# Autodesk Inventor assembly: bike
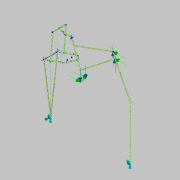
[picture p0: Inventor's stored thumbnail of the model, 180x180]
Saved by Autodesk Inventor 2021 (Build 250183000, 183)
## iProperties
RuleStatus: InUse
Created: 2020-04-29
Part Number: bike
Document SubType Name: Assembly
Designer: Hannah
Mass: 8583.94 g
Surface Area: 13590.5 cm^2
Volume: 2798.24 cm^3
Density: 3.06762 g/cm^3
Author: Hannah
## Documents named in this file (29)
- \\Mac\Home\Documents\GitHub\AdjustaBike-2.0\CAD\bike.iam
- \\Mac\Home\Documents\GitHub\AdjustaBike-2.0\CAD\prelim bike geo.ipt
- \\Mac\Home\Documents\GitHub\AdjustaBike-2.0\CAD\bottom bracket.ipt
- \\Mac\Home\Documents\GitHub\AdjustaBike-2.0\CAD\L10-7.ipt
- \\Mac\Home\Documents\GitHub\AdjustaBike-2.0\CAD\tube-07.ipt
- \\Mac\Home\Documents\GitHub\AdjustaBike-2.0\CAD\tube-08.ipt
- \\Mac\Home\Documents\GitHub\AdjustaBike-2.0\CAD\tube-09.ipt
- \\Mac\Home\Documents\GitHub\AdjustaBike-2.0\CAD\tube-11.ipt
- \\Mac\Home\Documents\GitHub\AdjustaBike-2.0\CAD\tube-12.ipt
- \\Mac\Home\Documents\GitHub\AdjustaBike-2.0\CAD\329-7.ipt
- \\Mac\Home\Documents\GitHub\AdjustaBike-2.0\CAD\head tube.ipt
- \\Mac\Home\Documents\GitHub\AdjustaBike-2.0\CAD\LM50-7.ipt
- \\Mac\Home\Documents\GitHub\AdjustaBike-2.0\CAD\LF50-6.ipt
- \\Mac\Home\Documents\GitHub\AdjustaBike-2.0\CAD\55-7.ipt
- \\Mac\Home\Documents\GitHub\AdjustaBike-2.0\CAD\L21-7.ipt
- \\Mac\Home\Documents\GitHub\AdjustaBike-2.0\CAD\tube-13.ipt
- \\Mac\Home\Documents\GitHub\AdjustaBike-2.0\CAD\LF50-7.ipt
- \\Mac\Home\Documents\GitHub\AdjustaBike-2.0\CAD\L10-6.ipt
- \\Mac\Home\Documents\GitHub\AdjustaBike-2.0\CAD\tube-14.ipt
- \\Mac\Home\Documents\GitHub\AdjustaBike-2.0\CAD\L114-6.ipt
- \\Mac\Home\Documents\GitHub\AdjustaBike-2.0\CAD\saddle.ipt
- \\Mac\Home\Documents\GitHub\AdjustaBike-2.0\CAD\M51-5.ipt
- \\Mac\Home\Documents\GitHub\AdjustaBike-2.0\CAD\link.ipt
- \\Mac\Home\Documents\GitHub\AdjustaBike-2.0\CAD\LM51-7.ipt
- \\Mac\Home\Documents\GitHub\AdjustaBike-2.0\CAD\main frame.ipt
- \\Mac\Home\Documents\GitHub\AdjustaBike-2.0\CAD\projectile.ipt
- \\Mac\Home\Documents\GitHub\AdjustaBike-2.0\CAD\dummy fork.ipt
- \\Mac\Home\Documents\GitHub\AdjustaBike-2.0\CAD\seatstays.ipt
- \\Mac\Home\Documents\GitHub\AdjustaBike-2.0\CAD\wheels.ipt
## Components (43 placed, 28 different names)
1. prelim bike geo:1 — Mate:1, Mate:2, Angle:1, Mate:41, Mate:140, Mate:149
2. main frame:1 — Mate:115, Mate:116, Mate:117, Mate:118, Mate:119, Mate:120, Mate:121, Mate:122, Mate:123, Mate:124, Mate:125, Mate:126, Mate:127, Mate:128, Mate:129, Mate:131, Mate:132, Mate:133, Mate:134, Mate:135, Mate:136, Mate:137, Mate:138, Mate:139, Mate:140, Mate:141, Mate:142, Mate:144, Flush:117, Flush:118, Flush:119, Flush:120, Flush:121, Flush:122, Flush:123, Flush:124, Flush:125
3. seatstays:1 — Flush:120, Flush:121, Flush:122, Mate:147, Mate:148
4. dummy fork:1 — Flush:117, Flush:118, Flush:119, Mate:149
5. projectile:1 — Mate:142, Mate:143, Mate:144, Mate:146
6. wheels:1 — Flush:123, Flush:124, Flush:125
7. bottom bracket:1 — Mate:4, Flush:1, Mate:5, Mate:6, Tangent:1, Mate:128, Mate:132, Mate:133
8. L10-7:1 — Mate:6, Flush:2, Mate:7, Mate:9
9. seat tube — Mate:7, Tangent:1, Flush:9, Angle:2, Mate:8, Angle:5, Mate:17, Tangent:7, Tangent:8, Mate:28, Mate:52, Flush:21, Mate:106, Mate:117
10. down tube — Flush:10, Angle:3, Tangent:2, Mate:11, Tangent:3, Angle:4, Mate:12, Mate:116
11. top tube — Mate:16, Tangent:4, Mate:18, Mate:115
12. seatstay:2 — Mate:45, Mate:47, Mate:82, Tangent:9, Mate:124
13. spacer:1 — Tangent:8, Mate:55, Mate:57, Mate:61, Mate:120
14. spacer:2 — Tangent:7, Mate:54, Mate:56, Mate:63, Mate:119
15. 329-7:1 — Mate:8, Mate:9, Mate:10, Angle:3, Tangent:2, Mate:11, Mate:53
16. 329-7:2 — Tangent:3, Angle:4, Mate:12, Mate:13, Mate:14, Flush:11
17. head tube:1 — Mate:14, Flush:11, Flush:12, Angle:5, Mate:15, Flush:13, Tangent:4, Mate:118, Mate:131
18. L10-7:2 — Mate:17, Mate:18
19. L10-7:3 — Mate:15, Flush:13, Flush:14, Mate:16, Mate:129
20. LM51-7:1 — Mate:28, Flush:16, Mate:69, Flush:20, Flush:21, Flush:22, Mate:107, Mate:110, Mate:111, Mate:112, Mate:113, Mate:114, Mate:138, Mate:139
21. LF50-6:2 — Mate:45, Mate:47, Angle:11, Mate:83, Flush:85
22. 55-7:1 — Mate:56, Mate:59, Mate:63, Mate:64
23. 55-7:2 — Mate:57, Mate:58, Mate:61, Mate:62
24. L21-7:1 — Mate:52, Mate:53, Mate:54, Mate:55, Mate:60
25. tube-13:1 — Mate:58, Mate:62, Angle:12, Mate:75, Mate:77, Mate:122
26. tube-13:2 — Mate:59, Mate:64, Angle:13, Mate:74, Mate:76, Mate:121
27. LF50-6:3 — Mate:69, Flush:20, Mate:98, Mate:99, Mate:108, Mate:109, Mate:126, Mate:141
28. LF50-7:1 — Mate:76, Mate:79, Mate:85, Mate:94, Mate:127, Mate:134
29. LF50-7:2 — Mate:77, Mate:78, Mate:85, Mate:86, Mate:135
30. LM50-7:3 — Mate:75, Mate:83, Flush:85, Mate:86
31. LM50-7:4 — Mate:74, Mate:94, Mate:95, Mate:96
32. L10-6:1 — Mate:82, Mate:89, Mate:137
33. tube-14:1 — Mate:89, Mate:90, Mate:92, Mate:100, Tangent:9, Mate:125, Mate:136, Mate:147, Mate:148
34. seatstay:1 — Mate:91, Mate:93, Mate:97, Mate:123
35. L10-6:3 — Mate:91, Mate:92
36. LF50-6:4 — Mate:93, Mate:95, Mate:96, Mate:97
37. L114-6:1 — Mate:98, Mate:99, Mate:100
38. saddle:1 — Mate:106, Flush:116
39. M51-5:1
40. link:1 — Mate:107, Mate:109
41. link:2 — Mate:111, Mate:113
42. link:3 — Mate:108, Mate:112
43. link:4 — Mate:110, Mate:114
## Relationships (143: Mate 105, Flush 23, Angle 8, Tangent 7)
- Mate:1: prelim bike geo:1
- Mate:2: prelim bike geo:1
- Mate:3
- Mate:4: bottom bracket:1
- Flush:1: bottom bracket:1
- Angle:1 (0 deg): prelim bike geo:1
- Mate:5: bottom bracket:1
- Mate:6: bottom bracket:1 ↔ L10-7:1
- Flush:2: L10-7:1
- Mate:7: L10-7:1 ↔ seat tube
- Tangent:1: bottom bracket:1 ↔ seat tube
- Flush:9: seat tube
- Angle:2 (-70 deg): seat tube
- Flush:10: down tube
- Mate:8: seat tube ↔ 329-7:1
- Mate:9 (5 mm): L10-7:1 ↔ 329-7:1
- Mate:10: 329-7:1
- Angle:3 (72 deg): down tube ↔ 329-7:1
- Tangent:2: down tube ↔ 329-7:1
- Mate:11: down tube ↔ 329-7:1
- Tangent:3: down tube ↔ 329-7:2
- Angle:4 (0 deg): down tube ↔ 329-7:2
- Mate:12: down tube ↔ 329-7:2
- Mate:13: 329-7:2
- Mate:14: 329-7:2 ↔ head tube:1
- Flush:11: 329-7:2 ↔ head tube:1
- Flush:12: head tube:1
- Angle:5 (0 deg): seat tube ↔ head tube:1
- Mate:15: head tube:1 ↔ L10-7:3
- Flush:13: head tube:1 ↔ L10-7:3
- Flush:14: L10-7:3
- Mate:16: top tube ↔ L10-7:3
- Tangent:4: top tube ↔ head tube:1
- Mate:17: seat tube ↔ L10-7:2
- Mate:18: top tube ↔ L10-7:2
- Tangent:7: seat tube ↔ spacer:2
- Tangent:8: seat tube ↔ spacer:1
- Mate:28: seat tube ↔ LM51-7:1
- Flush:16: LM51-7:1
- Mate:41: prelim bike geo:1
- Mate:45: seatstay:2 ↔ LF50-6:2
- Mate:47: seatstay:2 ↔ LF50-6:2
- Angle:11 (0 deg): LF50-6:2
- Mate:52: seat tube ↔ L21-7:1
- Mate:53 (5 mm): 329-7:1 ↔ L21-7:1
- Mate:54: spacer:2 ↔ L21-7:1
- Mate:55: spacer:1 ↔ L21-7:1
- Mate:56: spacer:2 ↔ 55-7:1
- Mate:57: spacer:1 ↔ 55-7:2
- Mate:58: 55-7:2 ↔ tube-13:1
- Mate:59: 55-7:1 ↔ tube-13:2
- Mate:60: L21-7:1
- Mate:61 (-30 mm): spacer:1 ↔ 55-7:2
- Mate:62 (-30 mm): 55-7:2 ↔ tube-13:1
- Mate:63 (-30 mm): spacer:2 ↔ 55-7:1
- Mate:64 (-30 mm): 55-7:1 ↔ tube-13:2
- Angle:12 (0 deg): tube-13:1
- Angle:13 (0 deg): tube-13:2
- Mate:69: LM51-7:1 ↔ LF50-6:3
- Flush:20: LM51-7:1 ↔ LF50-6:3
- Flush:21: seat tube ↔ LM51-7:1
- Mate:74: tube-13:2 ↔ LM50-7:4
- Mate:75: tube-13:1 ↔ LM50-7:3
- Mate:76: tube-13:2 ↔ LF50-7:1
- Mate:77: tube-13:1 ↔ LF50-7:2
- Mate:78: LF50-7:2
- Mate:79: LF50-7:1
- Flush:22: LM51-7:1
- Mate:82: seatstay:2 ↔ L10-6:1
- Mate:83: LF50-6:2 ↔ LM50-7:3
- Flush:85: LF50-6:2 ↔ LM50-7:3
- Mate:85: LF50-7:1 ↔ LF50-7:2
- Mate:86 (5 mm): LF50-7:2 ↔ LM50-7:3
- Mate:89: L10-6:1 ↔ tube-14:1
- Mate:90: tube-14:1
- Mate:91: seatstay:1 ↔ L10-6:3
- Mate:92: tube-14:1 ↔ L10-6:3
- Mate:93: seatstay:1 ↔ LF50-6:4
- Mate:94 (5 mm): LF50-7:1 ↔ LM50-7:4
- Mate:95: LM50-7:4 ↔ LF50-6:4
- Mate:96: LM50-7:4 ↔ LF50-6:4
- Mate:97: seatstay:1 ↔ LF50-6:4
- Mate:98: LF50-6:3 ↔ L114-6:1
- Mate:99: LF50-6:3 ↔ L114-6:1
- Mate:100: tube-14:1 ↔ L114-6:1
- Tangent:9: seatstay:2 ↔ tube-14:1
- [Mate]: saddle:1 ↔ M51-5:1
- [Mate]: M51-5:1 ↔ link:3
- [Mate]: M51-5:1 ↔ link:4
- [Mate]: M51-5:1 ↔ link:2
- [Mate]: M51-5:1 ↔ link:1
- Mate:106: seat tube ↔ saddle:1
- Mate:107: LM51-7:1 ↔ link:1
- Mate:108: LF50-6:3 ↔ link:3
- Mate:109: LF50-6:3 ↔ link:1
- Mate:110: LM51-7:1 ↔ link:4
- Mate:111: LM51-7:1 ↔ link:2
- Mate:112: LM51-7:1 ↔ link:3
- Mate:113: LM51-7:1 ↔ link:2
- Mate:114: LM51-7:1 ↔ link:4
- Flush:116: saddle:1
- Mate:115: main frame:1 ↔ top tube
- Mate:116: main frame:1 ↔ down tube
- Mate:117: main frame:1 ↔ seat tube
- Mate:118: main frame:1 ↔ head tube:1
- Mate:119: main frame:1 ↔ spacer:2
- Mate:120: main frame:1 ↔ spacer:1
- Mate:121: main frame:1 ↔ tube-13:2
- Mate:122: main frame:1 ↔ tube-13:1
- Mate:123: main frame:1 ↔ seatstay:1
- Mate:124: main frame:1 ↔ seatstay:2
- Mate:125: main frame:1 ↔ tube-14:1
- Mate:126: main frame:1 ↔ LF50-6:3
- Mate:127: main frame:1 ↔ LF50-7:1
- Mate:128: main frame:1 ↔ bottom bracket:1
- Mate:129: main frame:1 ↔ L10-7:3
- Mate:131: main frame:1 ↔ head tube:1
- Mate:132: main frame:1 ↔ bottom bracket:1
- Mate:133: main frame:1 ↔ bottom bracket:1
- Mate:134: main frame:1 ↔ LF50-7:1
- Mate:135: main frame:1 ↔ LF50-7:2
- Mate:136: main frame:1 ↔ tube-14:1
- Mate:137: main frame:1 ↔ L10-6:1
- Mate:138: main frame:1 ↔ LM51-7:1
- Mate:139: main frame:1 ↔ LM51-7:1
- Mate:140: prelim bike geo:1 ↔ main frame:1
- Mate:141: main frame:1 ↔ LF50-6:3
- Mate:142: main frame:1 ↔ projectile:1
- Mate:143: projectile:1
- Mate:144 (180 mm): main frame:1 ↔ projectile:1
- Mate:146: projectile:1
- Flush:117: main frame:1 ↔ dummy fork:1
- Flush:118: main frame:1 ↔ dummy fork:1
- Flush:119: main frame:1 ↔ dummy fork:1
- Flush:120: main frame:1 ↔ seatstays:1
- Flush:121: main frame:1 ↔ seatstays:1
- Flush:122: main frame:1 ↔ seatstays:1
- Mate:147: seatstays:1 ↔ tube-14:1
- Mate:148: seatstays:1 ↔ tube-14:1
- Mate:149: prelim bike geo:1 ↔ dummy fork:1
- Flush:123: main frame:1 ↔ wheels:1
- Flush:124: main frame:1 ↔ wheels:1
- Flush:125: main frame:1 ↔ wheels:1
## Named parameters: Lst = 440 mm, Sst = 7, Ldt = 500 mm, Sdt = 7, Ltt = 516 mm, Stt = 7, Lcs = 400 mm, Scs = 6, Lss = 230 mm, Sss = 6, Lsp = 75 mm, Ssp = 7, Lcsn = 170 mm, Scsn = 7, Lspn = 240 mm, d166_d164 = 0 mm
